# Autodesk Inventor assembly: EPS
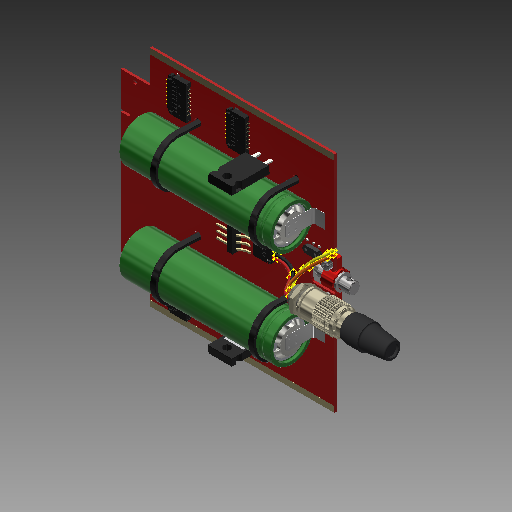
[picture p0: Inventor's stored thumbnail of the model, 512x512]
Saved by Autodesk Inventor 2018 (Build 220112000, 112)
## iProperties
Created: 2018-05-29
Part Number: EPS
Document SubType Name: Assembly
Designer: Bradley
Author: Bradley
## Documents named in this file (21)
- D:\Users\Bradley\Documents\CougsInSpace\CougSat1-Hardware\CougSat1-PowerBoard\CADModel\Native\EPS.iam
- D:\Users\Bradley\Documents\CougsInSpace\CougSat1-Hardware\CougSat1-PowerBoard\CADModel\Native\EPS_PCB.ipt
- D:\Users\Bradley\Documents\CougsInSpace\Resources\ComponentModels\Hardware\Pin_RBF.ipt
- D:\Users\Bradley\Documents\CougsInSpace\Resources\ComponentModels\Electronics\Switch_Micro-L.iam
- D:\Users\Bradley\Documents\CougsInSpace\Resources\ComponentModels\Electronics\Battery_18650.ipt
- D:\Users\Bradley\Documents\CougsInSpace\Resources\ComponentModels\Connectors\PicoLock--J-7.ipt
- D:\Users\Bradley\Documents\CougsInSpace\Resources\ComponentModels\Connectors\PicoLock--J-4.ipt
- D:\Users\Bradley\Documents\CougsInSpace\Resources\ComponentModels\Connectors\PicoLock--P-4.ipt
- D:\Users\Bradley\Documents\CougsInSpace\Resources\ComponentModels\Connectors\PicoLock--P-7.ipt
- D:\Users\Bradley\Documents\CougsInSpace\CougSat1-Hardware\CougSat1-PowerBoard\CADModel\Native\EPS_RBFPinHolder.ipt
- D:\Users\Bradley\Documents\CougsInSpace\Resources\ComponentModels\Fasteners\Bolt_M2x0.4_4mm_SH.ipt
- D:\Users\Bradley\Documents\CougsInSpace\CougSat1-Hardware\CougSat1-PowerBoard\CADModel\Native\EPS_SwitchNut.ipt
- D:\Users\Bradley\Documents\CougsInSpace\Resources\ComponentModels\Fasteners\Bolt_M1.6x0.35_5mm_SH.ipt
- D:\Users\Bradley\Documents\CougsInSpace\Resources\ComponentModels\Electronics\Resistor_TH-TO220.ipt
- D:\Users\Bradley\Documents\CougsInSpace\CougSat1-Hardware\CougSat1-PowerBoard\CADModel\Native\EPS_BatteryTab.ipt
- D:\Users\Bradley\Documents\CougsInSpace\CougSat1-Hardware\CougSat1-PowerBoard\CADModel\Native\EPS_BatteyTie.ipt
- D:\Users\Bradley\Documents\CougsInSpace\Resources\ComponentModels\Connectors\HR10A-7R-4P.ipt
- D:\Users\Bradley\Documents\CougsInSpace\Resources\ComponentModels\Connectors\HR10A-7P-4S.ipt
- D:\Users\Bradley\Documents\CougsInSpace\Resources\ComponentModels\Fasteners\Nut_M8x0.5_2mm.ipt
- D:\Users\Bradley\Documents\CougsInSpace\CougSat1-Hardware\CougSat1-PowerBoard\CADModel\Native\EPS\AIP\Cable and Harness\EPS.Harness.iam
- D:\Users\Bradley\Documents\CougsInSpace\Resources\ComponentModels\Connectors\SMD2.54-1x06-R.ipt
## Components (36 placed, 20 different names)
1. EPS_PCB:1 — Angle:1, Flush:1, Flush:2, Mate:14, Mate:15, Mate:16, Mate:17, Mate:18, Mate:19, Insert:4, Insert:5, Insert:6, Insert:7, Insert:8, Insert:9, Insert:10, Insert:11, Mate:22, Mate:23, Mate:24, Mate:25, Mate:26, Mate:35, Mate:36, Mate:37, Mate:38, Mate:45, Mate:46, Mate:47, Mate:48, Mate:49, Mate:50, Mate:51, Mate:52, Flush:23, Mate:55, Mate:56, Mate:57, Flush:28
2. EPS_RBFPinHolder:1 — Insert:3, Insert:4, Insert:9
3. EPS_SwitchNut:1 — Insert:10, Insert:11
4. EPS.Harness [sub-assembly]
5. HR10A-7R-4P:1 — Insert:14, Flush:20, Mate:53, Flush:22, Mate:54, Mate:55
6. HR10A-7P-4S:1 — Insert:14, Flush:20
7. PicoLock--J-4:1 — Flush:5, Mate:4, Mate:5, Mate:18, Mate:20, Mate:56
8. PicoLock--J-7:1 — Flush:6, Mate:6, Mate:7, Mate:14, Flush:14, Flush:24
9. PicoLock--J-7:2 — Mate:15, Flush:15, Flush:25
10. PicoLock--J-7:3 — Mate:16, Flush:14, Mate:23, Flush:26
11. PicoLock--J-7:4 — Mate:17, Flush:15, Mate:24, Flush:27
12. PicoLock--P-4:1 — Flush:5, Mate:4, Mate:5
13. PicoLock--P-7:1 — Flush:6, Mate:6, Mate:7
14. PicoLock--P-7:2
15. PicoLock--P-7:3
16. PicoLock--P-7:4
17. SMD2.54-1x06-R:1 — Mate:57, Mate:58, Flush:28
18. Battery_18650:1 — Flush:1, Flush:4, Flush:17, Mate:30, Mate:32, Mate:33, Mate:39, Flush:18, Mate:41, Mate:42
19. Battery_18650:2 — Flush:2, Flush:3, Mate:27, Mate:29, Mate:31, Mate:34, Mate:40, Flush:19, Mate:43, Mate:44
20. EPS_BatteryTab:1 — Mate:32, Mate:38, Mate:39
21. EPS_BatteryTab:2 — Mate:33, Mate:36, Flush:18
22. EPS_BatteryTab:3 — Mate:31, Mate:37, Mate:40
23. EPS_BatteryTab:4 — Mate:34, Mate:35, Flush:19
24. Resistor_TH-TO220:1 — Mate:22, Flush:17, Mate:25, Mate:28
25. Resistor_TH-TO220:2 — Mate:26, Mate:27, Mate:28
26. Switch_Micro-L:1 [sub-assembly] — Angle:1, Mate:19, Insert:5, Insert:6, Insert:12, Insert:13
27. Bolt_M1.6x0.35_5mm_SH:1 — Insert:12
28. Bolt_M1.6x0.35_5mm_SH:2 — Insert:13
29. Bolt_M2x0.4_4mm_SH:1 — Insert:7
30. Bolt_M2x0.4_4mm_SH:2 — Insert:8
31. EPS_BatteyTie:1 — Mate:41, Mate:47, Mate:49
32. EPS_BatteyTie:2 — Mate:42, Mate:48, Mate:50
33. EPS_BatteyTie:3 — Mate:43, Mate:45, Mate:51
34. EPS_BatteyTie:4 — Mate:44, Mate:46, Mate:52
35. Nut_M8x0.5_2mm:1 — Mate:54, Flush:23
36. Pin_RBF:1 — Insert:3
## Relationships (89: Mate 54, Flush 22, Insert 12, Angle 1)
- Angle:1 (0 deg): EPS_PCB:1 ↔ Switch_Micro-L:1
- Flush:1 (-9.15 mm): EPS_PCB:1 ↔ Battery_18650:1
- Flush:2 (-9.15 mm): EPS_PCB:1 ↔ Battery_18650:2
- Flush:3 (-50 mm): Battery_18650:2
- Flush:4 (-50 mm): Battery_18650:1
- Flush:5: PicoLock--J-4:1 ↔ PicoLock--P-4:1
- Mate:4: PicoLock--J-4:1 ↔ PicoLock--P-4:1
- Mate:5 (0.025 mm): PicoLock--J-4:1 ↔ PicoLock--P-4:1
- Flush:6: PicoLock--J-7:1 ↔ PicoLock--P-7:1
- Mate:6: PicoLock--J-7:1 ↔ PicoLock--P-7:1
- Mate:7 (0.025 mm): PicoLock--J-7:1 ↔ PicoLock--P-7:1
- [Flush]: PicoLock--J-7:2 ↔ PicoLock--P-7:2
- [Mate]: PicoLock--J-7:2 ↔ PicoLock--P-7:2
- [Mate] (0.025 mm): PicoLock--J-7:2 ↔ PicoLock--P-7:2
- [Flush]: PicoLock--J-7:3 ↔ PicoLock--P-7:3
- [Mate]: PicoLock--J-7:3 ↔ PicoLock--P-7:3
- [Mate] (0.025 mm): PicoLock--J-7:3 ↔ PicoLock--P-7:3
- [Flush]: PicoLock--J-7:4 ↔ PicoLock--P-7:4
- [Mate]: PicoLock--J-7:4 ↔ PicoLock--P-7:4
- [Mate] (0.025 mm): PicoLock--J-7:4 ↔ PicoLock--P-7:4
- Mate:14: EPS_PCB:1 ↔ PicoLock--J-7:1
- Mate:15: EPS_PCB:1 ↔ PicoLock--J-7:2
- Mate:16: EPS_PCB:1 ↔ PicoLock--J-7:3
- Mate:17: EPS_PCB:1 ↔ PicoLock--J-7:4
- Mate:18: EPS_PCB:1 ↔ PicoLock--J-4:1
- Flush:14: PicoLock--J-7:1 ↔ PicoLock--J-7:3
- Flush:15: PicoLock--J-7:2 ↔ PicoLock--J-7:4
- Mate:19 (-8.75 mm): EPS_PCB:1 ↔ Switch_Micro-L:1
- Insert:3: EPS_RBFPinHolder:1 ↔ Pin_RBF:1
- Insert:4: EPS_PCB:1 ↔ EPS_RBFPinHolder:1
- Insert:5: EPS_PCB:1 ↔ Switch_Micro-L:1
- Insert:6: EPS_PCB:1 ↔ Switch_Micro-L:1
- Insert:7: EPS_PCB:1 ↔ Bolt_M2x0.4_4mm_SH:1
- Insert:8: EPS_PCB:1 ↔ Bolt_M2x0.4_4mm_SH:2
- Insert:9: EPS_PCB:1 ↔ EPS_RBFPinHolder:1
- Insert:10: EPS_PCB:1 ↔ EPS_SwitchNut:1
- Insert:11: EPS_PCB:1 ↔ EPS_SwitchNut:1
- Insert:12: Switch_Micro-L:1 ↔ Bolt_M1.6x0.35_5mm_SH:1
- Insert:13: Switch_Micro-L:1 ↔ Bolt_M1.6x0.35_5mm_SH:2
- Mate:20: PicoLock--J-4:1
- Mate:22: EPS_PCB:1 ↔ Resistor_TH-TO220:1
- Flush:17 (9.15 mm): Battery_18650:1 ↔ Resistor_TH-TO220:1
- Mate:23 (-30 mm): EPS_PCB:1 ↔ PicoLock--J-7:3
- Mate:24 (-55 mm): EPS_PCB:1 ↔ PicoLock--J-7:4
- Mate:25 (-62 mm): EPS_PCB:1 ↔ Resistor_TH-TO220:1
- Mate:26: EPS_PCB:1 ↔ Resistor_TH-TO220:2
- Mate:27 (9.15 mm): Battery_18650:2 ↔ Resistor_TH-TO220:2
- Mate:28: Resistor_TH-TO220:1 ↔ Resistor_TH-TO220:2
- Mate:29 (-21 mm): Battery_18650:2
- Mate:30 (21 mm): Battery_18650:1
- Mate:31: Battery_18650:2 ↔ EPS_BatteryTab:3
- Mate:32: Battery_18650:1 ↔ EPS_BatteryTab:1
- Mate:33: Battery_18650:1 ↔ EPS_BatteryTab:2
- Mate:34: Battery_18650:2 ↔ EPS_BatteryTab:4
- Mate:35: EPS_PCB:1 ↔ EPS_BatteryTab:4
- Mate:36: EPS_PCB:1 ↔ EPS_BatteryTab:2
- Mate:37: EPS_PCB:1 ↔ EPS_BatteryTab:3
- Mate:38: EPS_PCB:1 ↔ EPS_BatteryTab:1
- Mate:39: Battery_18650:1 ↔ EPS_BatteryTab:1
- Flush:18: Battery_18650:1 ↔ EPS_BatteryTab:2
- Mate:40: Battery_18650:2 ↔ EPS_BatteryTab:3
- Flush:19: Battery_18650:2 ↔ EPS_BatteryTab:4
- Mate:41: Battery_18650:1 ↔ EPS_BatteyTie:1
- Mate:42: Battery_18650:1 ↔ EPS_BatteyTie:2
- Mate:43: Battery_18650:2 ↔ EPS_BatteyTie:3
- Mate:44: Battery_18650:2 ↔ EPS_BatteyTie:4
- Mate:45: EPS_PCB:1 ↔ EPS_BatteyTie:3
- Mate:46: EPS_PCB:1 ↔ EPS_BatteyTie:4
- Mate:47: EPS_PCB:1 ↔ EPS_BatteyTie:1
- Mate:48: EPS_PCB:1 ↔ EPS_BatteyTie:2
- Mate:49: EPS_PCB:1 ↔ EPS_BatteyTie:1
- Mate:50: EPS_PCB:1 ↔ EPS_BatteyTie:2
- Mate:51: EPS_PCB:1 ↔ EPS_BatteyTie:3
- Mate:52: EPS_PCB:1 ↔ EPS_BatteyTie:4
- Insert:14: HR10A-7R-4P:1 ↔ HR10A-7P-4S:1
- Flush:20: HR10A-7R-4P:1 ↔ HR10A-7P-4S:1
- Mate:53 (13 mm): HR10A-7R-4P:1
- Flush:22: HR10A-7R-4P:1
- Mate:54: HR10A-7R-4P:1 ↔ Nut_M8x0.5_2mm:1
- Flush:23: EPS_PCB:1 ↔ Nut_M8x0.5_2mm:1
- Mate:55 (1.7 mm): EPS_PCB:1 ↔ HR10A-7R-4P:1
- Mate:56 (-33 mm): EPS_PCB:1 ↔ PicoLock--J-4:1
- Flush:24 (-36.75 mm): PicoLock--J-7:1
- Flush:25 (-36.75 mm): PicoLock--J-7:2
- Flush:26 (36.75 mm): PicoLock--J-7:3
- Flush:27 (36.75 mm): PicoLock--J-7:4
- Mate:57: EPS_PCB:1 ↔ SMD2.54-1x06-R:1
- Mate:58 (6.35 mm): SMD2.54-1x06-R:1
- Flush:28 (50 mm): EPS_PCB:1 ↔ SMD2.54-1x06-R:1
## Named parameters: d15_d12 = 0 mm, d16_d13 = 0 mm, d17_d14 = 0.025 mm, d18_d12 = 0 mm, d19_d13 = 0 mm, d20_d14 = 0.025 mm, d21_d12 = 0 mm, d22_d13 = 0 mm, d23_d14 = 0.025 mm
